# Autodesk Inventor assembly: spojkasgondolounova
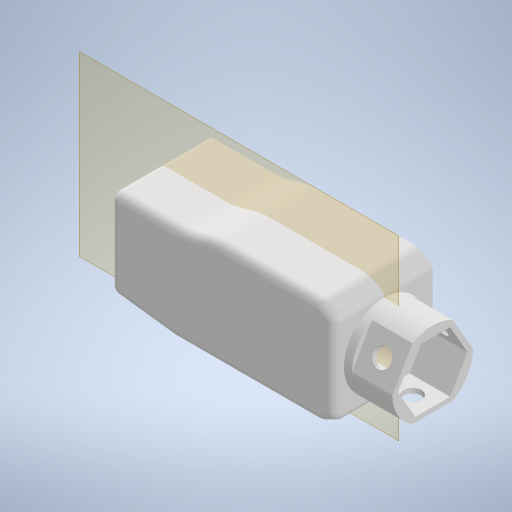
[picture p0: Inventor's stored thumbnail of the model, 512x512]
Saved by Autodesk Inventor 2023 (Build 270158000, 158)
## iProperties
Created: 2023-12-26
Part Number: spojkasgondolounova
Document SubType Name: Assembly
Designer: alexa
Author: alexa
## Documents named in this file (3)
- C:\Users\alexa\OneDrive - Stredni prumyslova skola\Desktop\Inventor\Vetrna elektrarna\spojkasgondolounova.iam
- C:\Users\alexa\OneDrive - Stredni prumyslova skola\Desktop\Inventor\Vetrna elektrarna\gondola.ipt
- C:\Users\alexa\OneDrive - Stredni prumyslova skola\Desktop\Inventor\Vetrna elektrarna\spojkaV2.ipt
## Components (2 placed, 2 different names)
1. gondola:1 — Mate:1, Mate:2
2. spojkaV2:1 — Mate:1, Mate:2
## Relationships (2: Mate 2)
- Mate:1: gondola:1 ↔ spojkaV2:1
- Mate:2: gondola:1 ↔ spojkaV2:1
